# Autodesk Inventor assembly: Ensamble
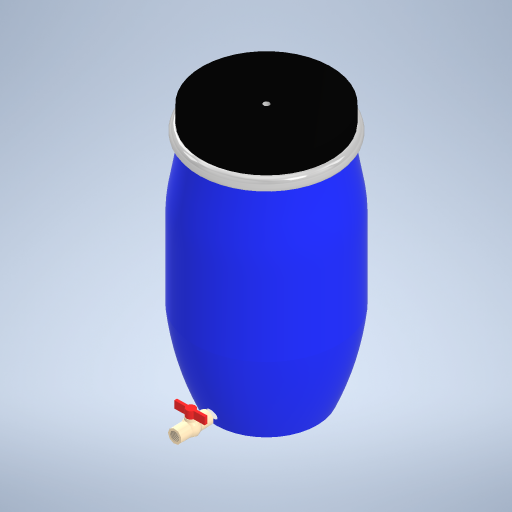
[picture p0: Inventor's stored thumbnail of the model, 512x512]
Saved by Autodesk Inventor 2024 (Build 280153000, 153)
## iProperties
Created: 2024-04-30
Part Number: Ensamble
Document SubType Name: Assembly
Designer: alexa
Author: alexa
## Documents named in this file (3)
- C:\Users\alexa\OneDrive\Escritorio\Biogas\Estructura\Ensamble.iam
- C:\Users\alexa\OneDrive\Escritorio\Biogas\Estructura\Contenedor.ipt
- C:\Users\alexa\OneDrive\Escritorio\Biogas\Estructura\LlaveDesecho.ipt
## Components (2 placed, 2 different names)
1. Contenedor:1 — Mate:2, Mate:5, Mate:6
2. LlaveDesecho:1 — Mate:5, Mate:6
## Relationships (3: Mate 3)
- Mate:2: Contenedor:1
- Mate:5: Contenedor:1 ↔ LlaveDesecho:1
- Mate:6: Contenedor:1 ↔ LlaveDesecho:1
